# Autodesk Inventor assembly: wire guidance wheel
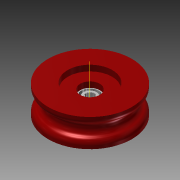
[picture p0: Inventor's stored thumbnail of the model, 180x180]
Saved by Autodesk Inventor 2013 (Build 170138000, 138)
## iProperties
Created: 2012-11-19
Part Number: wire guidance wheel
Document SubType Name: Assembly
Designer: Nico
Author: Nico
## Documents named in this file (4)
- D:\Documents\Inventor\Coil winder\IAM files\wire guidance wheel.iam
- D:\Documents\Inventor\Coil winder\IPT files\Wire guidance wheelV2.ipt
- D:\Documents\Inventor\Coil winder\IPT files\Bearring cap 8mm.ipt
- D:\Documents\Inventor\Content Center Files\R2013\en-US\ISO 1224 (I) M\ISO 1224 - 39 - 3 x 8 x 4.ipt
## Components (3 placed, 3 different names)
1. Wire guidance wheelV2:1 — Mate:1, Mate:2, Mate:3, Mate:4
2. Bearring cap 8mm:1 — Mate:3, Mate:4
3. ISO 1224 (I) (Metric) 39 - 3 x 8 x 4:1 — Mate:1, Mate:2
## Relationships (4: Mate 4)
- Mate:1: Wire guidance wheelV2:1 ↔ ISO 1224 (I) (Metric) 39 - 3 x 8 x 4:1
- Mate:2: Wire guidance wheelV2:1 ↔ ISO 1224 (I) (Metric) 39 - 3 x 8 x 4:1
- Mate:3: Wire guidance wheelV2:1 ↔ Bearring cap 8mm:1
- Mate:4 (0.2 mm): Wire guidance wheelV2:1 ↔ Bearring cap 8mm:1
